# Autodesk Inventor assembly: Arm for Gen 2
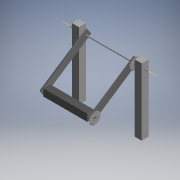
[picture p0: Inventor's stored thumbnail of the model, 180x180]
Saved by Autodesk Inventor 2019 (Build 230136000, 136)
## iProperties
Part Number: Arm for Gen 2
Document SubType Name: Assembly
Designer: Delta
Author: Delta
## Documents named in this file (7)
- C:\Robotics\2019-20_CAD\Collection\Arm for Gen 2.iam
- C:\Robotics\2019-20_CAD\Collection\30x30 pillars.ipt
- C:\Robotics\2019-20_CAD\Collection\12 Inch Hex Axle.ipt
- C:\Robotics\COTSParts\Sprockets - AndyMark\615106.ipt
- C:\Robotics\2019-20_CAD\Collection\bar arms.ipt
- C:\Robotics\2019-20_CAD\Collection\Claw holding bars.ipt
- C:\Robotics\2019-20_CAD\Collection\Spacer .25D .2H.ipt
## Components (12 placed, 6 different names)
1. 30x30 pillars:1 — Mate:2, Flush:2, Mate:11, Mate:21
2. 30x30 pillars:2 — Mate:3, Flush:2, Mate:11, Angle:1, Mate:18
3. 12 Inch Hex Axle:1 — Mate:2, Mate:3, Mate:5, Mate:6, Mate:8, Mate:23
4. 615106:1 — Mate:5, Mate:18, Mate:19, Mate:27
5. bar arms:1 — Mate:6, Flush:5, Mate:21, Mate:24
6. bar arms:2 — Mate:8, Flush:5, Mate:14, Mate:15, Mate:16, Mate:19, Mate:20, Mate:25
7. Claw holding bars:1 — Mate:14, Mate:15, Angle:1, Mate:26, Mate:28
8. 615106:2 — Mate:16, Mate:20, Mate:29, Mate:30
9. Spacer .25D .2H:1 — Mate:29, Mate:30
10. Spacer .25D .2H:2 — Mate:25, Mate:26
11. Spacer .25D .2H:3 — Mate:23, Mate:27
12. Spacer .25D .2H:4 — Mate:24, Mate:28
## Relationships (24: Mate 21, Flush 2, Angle 1)
- Mate:2: 30x30 pillars:1 ↔ 12 Inch Hex Axle:1
- Mate:3: 30x30 pillars:2 ↔ 12 Inch Hex Axle:1
- Flush:2: 30x30 pillars:1 ↔ 30x30 pillars:2
- Mate:5: 12 Inch Hex Axle:1 ↔ 615106:1
- Mate:6: 12 Inch Hex Axle:1 ↔ bar arms:1
- Mate:8: 12 Inch Hex Axle:1 ↔ bar arms:2
- Flush:5: bar arms:1 ↔ bar arms:2
- Mate:11 (254 mm): 30x30 pillars:1 ↔ 30x30 pillars:2
- Mate:14: bar arms:2 ↔ Claw holding bars:1
- Mate:15 (5.08 mm): bar arms:2 ↔ Claw holding bars:1
- Angle:1 (0 deg): 30x30 pillars:2 ↔ Claw holding bars:1
- Mate:16: bar arms:2 ↔ 615106:2
- Mate:18 (11.43 mm): 30x30 pillars:2 ↔ 615106:1
- Mate:19 (5.08 mm): 615106:1 ↔ bar arms:2
- Mate:20 (5.08 mm): bar arms:2 ↔ 615106:2
- Mate:21 (11.43 mm): 30x30 pillars:1 ↔ bar arms:1
- Mate:23: 12 Inch Hex Axle:1 ↔ Spacer .25D .2H:3
- Mate:24: bar arms:1 ↔ Spacer .25D .2H:4
- Mate:25: bar arms:2 ↔ Spacer .25D .2H:2
- Mate:26: Claw holding bars:1 ↔ Spacer .25D .2H:2
- Mate:27: 615106:1 ↔ Spacer .25D .2H:3
- Mate:28: Claw holding bars:1 ↔ Spacer .25D .2H:4
- Mate:29: 615106:2 ↔ Spacer .25D .2H:1
- Mate:30: 615106:2 ↔ Spacer .25D .2H:1
